# Autodesk Inventor assembly: A001-Bras-Optique
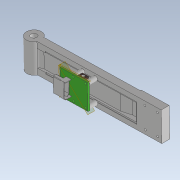
[picture p0: Inventor's stored thumbnail of the model, 180x180]
Saved by Autodesk Inventor 2020 (Build 240168000, 168)
## iProperties
Created: 2021-07-23
Part Number: A001-Bras-Optique
Document SubType Name: Assembly
Designer: gregory.trottet
Author: gregory.trottet
## Documents named in this file (4)
- C:\Users\gregory.trottet\Desktop\PROJECTS\31-Projet-Martial\Bras\A001-Bras-Optique.iam
- C:\Users\gregory.trottet\Desktop\PROJECTS\31-Projet-Martial\Bras\P001-Bras.ipt
- C:\Users\gregory.trottet\Desktop\PROJECTS\31-Projet-Martial\Bras\F001-PCB1.ipt
- C:\Users\gregory.trottet\Desktop\PROJECTS\31-Projet-Martial\Bras\P003-Entretoise-M2.ipt
## Components (6 placed, 3 different names)
1. P001-Bras:1 — Mate:1, Mate:2, Mate:3, Mate:4, Mate:5, Mate:6, Mate:7, Mate:8
2. F001-PCB1:1 — Mate:9, Mate:10, Mate:11
3. P003-Entretoise-M2:1 — Mate:3, Mate:4, Mate:10
4. P003-Entretoise-M2:2 — Mate:1, Mate:2
5. P003-Entretoise-M2:3 — Mate:5, Mate:6, Mate:9
6. P003-Entretoise-M2:4 — Mate:7, Mate:8, Mate:11
## Relationships (11: Mate 11)
- Mate:1: P001-Bras:1 ↔ P003-Entretoise-M2:2
- Mate:2: P001-Bras:1 ↔ P003-Entretoise-M2:2
- Mate:3: P001-Bras:1 ↔ P003-Entretoise-M2:1
- Mate:4: P001-Bras:1 ↔ P003-Entretoise-M2:1
- Mate:5: P001-Bras:1 ↔ P003-Entretoise-M2:3
- Mate:6: P001-Bras:1 ↔ P003-Entretoise-M2:3
- Mate:7: P001-Bras:1 ↔ P003-Entretoise-M2:4
- Mate:8: P001-Bras:1 ↔ P003-Entretoise-M2:4
- Mate:9: F001-PCB1:1 ↔ P003-Entretoise-M2:3
- Mate:10: F001-PCB1:1 ↔ P003-Entretoise-M2:1
- Mate:11: F001-PCB1:1 ↔ P003-Entretoise-M2:4
